# Autodesk Inventor assembly: RollingSquareC1
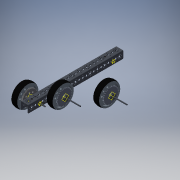
[picture p0: Inventor's stored thumbnail of the model, 180x180]
Saved by Autodesk Inventor 2016 (Build 200138000, 138)
## iProperties
Created: 2015-08-30
Part Number: RollingSquareC1
Document SubType Name: Assembly
Designer: Tim
Author: Tim
## Documents named in this file (5)
- C:\Users\Tim\Documents\GitHub\phi_robotics\3d-models\FTC_Tetrix_KOP_Block_Party\Tim Bloot Designs\RollingSquareC1.iam
- C:\Users\Tim\Documents\GitHub\phi_robotics\3d-models\FTC_Tetrix_KOP_Block_Party\Tetrix_Kit_FTC\Autodesk Inventor Files\tetrix_c_channel-5.ipt
- C:\Users\Tim\Documents\GitHub\phi_robotics\3d-models\FTC_Tetrix_KOP_Block_Party\Tetrix_Kit_FTC\Autodesk Inventor Files\tetrix_bushing.ipt
- C:\Users\Tim\Documents\GitHub\phi_robotics\3d-models\FTC_Tetrix_KOP_Block_Party\Tetrix_Kit_FTC\Autodesk Inventor Files\tetrix_739092_2012.iam
- C:\Users\Tim\Documents\GitHub\phi_robotics\3d-models\FTC_Tetrix_KOP_Block_Party\Tim Bloot Designs\WheelNChainGear.iam
## Components (9 placed, 4 different names)
1. tetrix_c_channel-5:1 — Rotational:3, Rotational:4, Rotational:6, Rotational:7
2. tetrix_bushing:3 — Rotational:3
3. tetrix_bushing:4 — Rotational:4, Rotational:9
4. tetrix_739092_2012:1 [sub-assembly] — Rigid:9
5. tetrix_bushing:5 — Rotational:6
6. tetrix_bushing:6 — Rotational:7, Rotational:8
7. tetrix_739092_2012:2 [sub-assembly] — Rigid:8
8. WheelNChainGear:1 [sub-assembly] — Rotational:8, Rigid:8
9. WheelNChainGear:2 [sub-assembly] — Rotational:9, Rigid:9
## Relationships (8: RevoluteJoint 6, WeldJoint 2)
- Rotational:3 [RevoluteJoint]: tetrix_c_channel-5:1 ↔ tetrix_bushing:3
- Rotational:4 [RevoluteJoint]: tetrix_c_channel-5:1 ↔ tetrix_bushing:4
- Rotational:6 [RevoluteJoint]: tetrix_c_channel-5:1 ↔ tetrix_bushing:5
- Rotational:7 [RevoluteJoint]: tetrix_c_channel-5:1 ↔ tetrix_bushing:6
- Rotational:8 [RevoluteJoint] (-25 mm): tetrix_bushing:6 ↔ WheelNChainGear:1
- Rigid:8 [WeldJoint] (-19 mm): tetrix_739092_2012:2 ↔ WheelNChainGear:1
- Rotational:9 [RevoluteJoint] (-25 mm): tetrix_bushing:4 ↔ WheelNChainGear:2
- Rigid:9 [WeldJoint] (-19 mm): tetrix_739092_2012:1 ↔ WheelNChainGear:2
